# Autodesk Inventor assembly: SHANK2
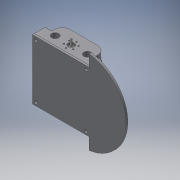
[picture p0: Inventor's stored thumbnail of the model, 180x180]
Saved by Autodesk Inventor 2017 (Build 210142000, 142)
## iProperties
Created: 2017-05-03
Part Number: SHANK2
Document SubType Name: Assembly
Designer: ANDRES
Author: ANDRES
## Documents named in this file (4)
- D:\MIS COSAS\Drive\Publica\UCABBOTS2017\Laberinto\Diseño Mecanico\SHANK2.iam
- D:\MIS COSAS\Drive\Publica\UCABBOTS2017\Laberinto\Diseño Mecanico\PCB_Final.ipt
- D:\MIS COSAS\Drive\Publica\UCABBOTS2017\Laberinto\Diseño Mecanico\Base_Motor_acrilico_15.ipt
- D:\MIS COSAS\Drive\Publica\UCABBOTS2017\Laberinto\Diseño Mecanico\Motor_Final.ipt
## Components (5 placed, 3 different names)
1. PCB_Final:1 — Mate:1, Mate:2, Mate:3, Flush:1, Mate:5, Flush:2, Mate:8
2. Base_Motor_acrilico_15:1 — Mate:2, Flush:2, Mate:8
3. Base_Motor_acrilico_15:2 — Mate:3, Flush:1, Mate:5, Cylindrical:1, Mate:7
4. Motor_Final:1 — Cylindrical:1, Mate:6, Cylindrical:2, Mate:7
5. Motor_Final:2 — Mate:6, Cylindrical:2
## Relationships (11: Mate 7, Flush 2, CylindricalJoint 2)
- Mate:1: PCB_Final:1
- Mate:2: PCB_Final:1 ↔ Base_Motor_acrilico_15:1
- Mate:3: PCB_Final:1 ↔ Base_Motor_acrilico_15:2
- Flush:1: PCB_Final:1 ↔ Base_Motor_acrilico_15:2
- Mate:5: PCB_Final:1 ↔ Base_Motor_acrilico_15:2
- Cylindrical:1: Base_Motor_acrilico_15:2 ↔ Motor_Final:1
- Mate:6: Motor_Final:1 ↔ Motor_Final:2
- Cylindrical:2: Motor_Final:1 ↔ Motor_Final:2
- Mate:7: Base_Motor_acrilico_15:2 ↔ Motor_Final:1
- Flush:2: PCB_Final:1 ↔ Base_Motor_acrilico_15:1
- Mate:8: PCB_Final:1 ↔ Base_Motor_acrilico_15:1
